# Autodesk Inventor assembly: CameraAndLightRingMount
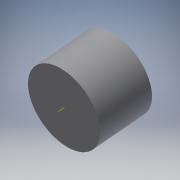
[picture p0: Inventor's stored thumbnail of the model, 180x180]
Saved by Autodesk Inventor 2019.1 (Build 231200000, 200)
## iProperties
Created: 2018-11-03
Part Number: CameraAndLightRingMount
Document SubType Name: Assembly
Designer: steele
Author: steele
## Documents named in this file (3)
- C:\git\CAD-Development\robSteele\CameraAndLightRingMount\CameraAndLightRingMount.iam
- C:\git\CAD-Development\robSteele\CameraAndLightRingMount\MountV01.ipt
- C:\git\CAD-Development\robSteele\CameraAndLightRingMount\fc18-097_RingLights.ipt
## Components (2 placed, 2 different names)
1. MountV01:1 — Mate:1, Mate:2
2. fc18-097_RingLights:1 — Mate:1, Mate:2
## Relationships (2: Mate 2)
- Mate:1: MountV01:1 ↔ fc18-097_RingLights:1
- Mate:2: MountV01:1 ↔ fc18-097_RingLights:1
